# Autodesk Inventor assembly: Tiger
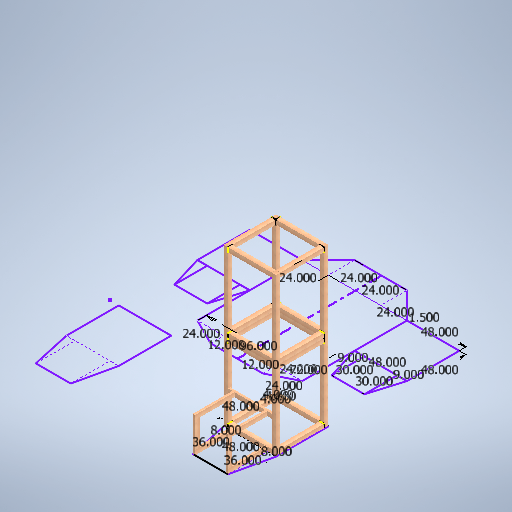
[picture p0: Inventor's stored thumbnail of the model, 512x512]
Saved by Autodesk Inventor 2025 (Build 290162000, 162)
## iProperties
Created: 2024-06-05
Part Number: Tiger
Document SubType Name: Assembly
Designer: Cupri
Mass: 180546 g
Surface Area: 136258 cm^2
Volume: 328266 cm^3
Density: 0.55 g/cm^3
Author: Cupri
## Documents named in this file (12)
- C:\Users\Cupri\OneDrive\Documents\TigerBurn\USCTigerBurn24\v1\Tiger.iam
- C:\Users\Cupri\OneDrive\Documents\TigerBurn\USCTigerBurn24\Standard Timber\4x4x72.ipt
- C:\Users\Cupri\OneDrive\Documents\TigerBurn\USCTigerBurn24\Standard Timber\4x4x40.ipt
- C:\Users\Cupri\OneDrive\Documents\TigerBurn\USCTigerBurn24\Standard Timber\2x4x36.ipt
- C:\Users\Cupri\OneDrive\Documents\TigerBurn\USCTigerBurn24\Standard Timber\2x4x40.ipt
- C:\Users\Cupri\OneDrive\Documents\TigerBurn\USCTigerBurn24\Standard Timber\2x4x24.ipt
- C:\Users\Cupri\OneDrive\Documents\TigerBurn\USCTigerBurn24\v1\Tiger\AIP\FEA\epzzwi8io.fins
- C:\Users\Cupri\OneDrive\Documents\TigerBurn\USCTigerBurn24\v1\Tiger\AIP\FEA\epzzwi8io.fsat
- C:\Users\Cupri\OneDrive\Documents\TigerBurn\USCTigerBurn24\v1\Tiger\AIP\FEA\epzzwi8io.ftes
- C:\Users\Cupri\OneDrive\Documents\TigerBurn\USCTigerBurn24\v1\Tiger\AIP\FEA\epzzwi8io.fwiz
- C:\Users\Cupri\OneDrive\Documents\TigerBurn\USCTigerBurn24\v1\Tiger\AIP\FEA\epzzwi8jk.fmsh
- C:\Users\Cupri\OneDrive\Documents\TigerBurn\USCTigerBurn24\v1\Tiger\AIP\FEA\epzzwi8jl.fres
## Components (31 placed, 5 different names)
1. 4x4x72:1 — Rigid:1, Rigid:3, Rigid:10, Rigid:11
2. 4x4x72:2 — Rigid:2, Rigid:4, Rigid:8
3. 4x4x40:1 — Rigid:1, Rigid:2
4. 4x4x40:2 — Rigid:3, Rigid:5
5. 4x4x40:3 — Rigid:6, Mate:5, Mate:6, Flush:4, Flush:5
6. 4x4x40:4 — Rigid:4, Rigid:7
7. 4x4x40:5 — Rigid:8
8. 4x4x40:6 — Rigid:9, Rigid:23
9. 4x4x40:7 — Rigid:11
10. 4x4x40:8 — Rigid:10
11. 4x4x72:3 — Rigid:5, Rigid:6, Rigid:9, Mate:4, Flush:3
12. 4x4x72:4 — Rigid:7, Mate:7
13. 4x4x72:5
14. 4x4x72:6
15. 4x4x40:9
16. 4x4x40:10
17. 4x4x40:11 — Rigid:23
18. 4x4x40:12
19. 4x4x40:13
20. 4x4x40:14
21. 4x4x40:15
22. 4x4x40:16
23. 4x4x72:7
24. 4x4x72:8
25. 2x4x40:1 — Mate:4, Flush:3, Mate:5, Mate:8, Flush:6, Mate:9, Flush:7
26. 2x4x36:1 — Mate:6, Flush:4, Rigid:24
27. 2x4x36:2 — Mate:8, Flush:6
28. 2x4x36:3 — Mate:9, Flush:7, Mate:10
29. 2x4x36:4 — Mate:7, Flush:5, Mate:10, Rigid:25
30. 2x4x24:1 — Rigid:24
31. 2x4x24:2 — Rigid:25
## Relationships (37: WeldJoint 25, Mate 7, Flush 5)
- Rigid:1 [WeldJoint]: 4x4x72:1 ↔ 4x4x40:1
- Rigid:2 [WeldJoint]: 4x4x72:2 ↔ 4x4x40:1
- Rigid:3 [WeldJoint]: 4x4x72:1 ↔ 4x4x40:2
- Rigid:4 [WeldJoint]: 4x4x72:2 ↔ 4x4x40:4
- Rigid:5 [WeldJoint]: 4x4x40:2 ↔ 4x4x72:3
- Rigid:6 [WeldJoint]: 4x4x40:3 ↔ 4x4x72:3
- Rigid:7 [WeldJoint]: 4x4x40:4 ↔ 4x4x72:4
- Rigid:8 [WeldJoint]: 4x4x72:2 ↔ 4x4x40:5
- Rigid:9 [WeldJoint]: 4x4x40:6 ↔ 4x4x72:3
- Rigid:10 [WeldJoint]: 4x4x72:1 ↔ 4x4x40:8
- Rigid:11 [WeldJoint]: 4x4x72:1 ↔ 4x4x40:7
- [WeldJoint]: 4x4x72:5 ↔ 4x4x40:9
- [WeldJoint]: 4x4x72:6 ↔ 4x4x40:9
- [WeldJoint]: 4x4x72:5 ↔ 4x4x40:10
- [WeldJoint]: 4x4x72:6 ↔ 4x4x40:12
- [WeldJoint]: 4x4x40:10 ↔ 4x4x72:7
- [WeldJoint]: 4x4x40:11 ↔ 4x4x72:7
- [WeldJoint]: 4x4x40:12 ↔ 4x4x72:8
- [WeldJoint]: 4x4x72:6 ↔ 4x4x40:13
- [WeldJoint]: 4x4x40:14 ↔ 4x4x72:7
- [WeldJoint]: 4x4x72:5 ↔ 4x4x40:16
- [WeldJoint]: 4x4x72:5 ↔ 4x4x40:15
- Rigid:23 [WeldJoint]: 4x4x40:6 ↔ 4x4x40:11
- Mate:4: 4x4x72:3 ↔ 2x4x40:1
- Flush:3: 4x4x72:3 ↔ 2x4x40:1
- Mate:5 (609.6 mm): 4x4x40:3 ↔ 2x4x40:1
- Mate:6 (101.6 mm): 4x4x40:3 ↔ 2x4x36:1
- Flush:4: 4x4x40:3 ↔ 2x4x36:1
- Mate:7 (101.6 mm): 4x4x72:4 ↔ 2x4x36:4
- Flush:5: 4x4x40:3 ↔ 2x4x36:4
- Mate:8 (101.6 mm): 2x4x40:1 ↔ 2x4x36:2
- Flush:6: 2x4x40:1 ↔ 2x4x36:2
- Mate:9: 2x4x40:1 ↔ 2x4x36:3
- Flush:7: 2x4x40:1 ↔ 2x4x36:3
- Mate:10: 2x4x36:3 ↔ 2x4x36:4
- Rigid:24 [WeldJoint]: 2x4x36:1 ↔ 2x4x24:1
- Rigid:25 [WeldJoint]: 2x4x36:4 ↔ 2x4x24:2
## Named parameters: d40_d29 = 0 mm, d41_d30 = 0 mm, d42_d31 = 0 mm, d43_d32 = 0 mm, d44_d33 = 0 mm, d45_d34 = 0 mm, d46_d35 = 0 mm, d47_d36 = 0 mm, d48_d37 = 0 mm, d49_d38 = 0 mm, d50_d39 = 0 mm, sa_0 = 22241.1
note: some values were not read from the file. Shown as the stored number, unit unknown: "sa_0".
